# Autodesk Inventor assembly: KS-14_SLow_10inch
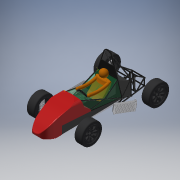
[picture p0: Inventor's stored thumbnail of the model, 180x180]
Saved by Autodesk Inventor 2018.1 (Build 221171000, 171)
## iProperties
Created: 2017-10-13
Part Number: KS-14_SLow_10inch
Material: 一般
Document SubType Name: Assembly
Designer: kuwano
Sending System: Autodesk Inventor 2018
Preprocessor: ST-DEVELOPER v16.13
Title: D:\kuwano\Documents\Inventor\KITformula\CFD_KS-14\KS-14\stl\final_assembly_2017_SuperUltraLow.stp
Author: kuwano
## Documents named in this file (15)
- D:\kuwano\Documents\Inventor\KITformula\KS-15_Aero_CAD\ks-14_slow\KS-14_SLow_10inch.iam
- D:\kuwano\Documents\Inventor\KITformula\KS-15_Aero_CAD\KS-14_SLow\parts\frame3kaiseki_retutch.ipt
- D:\kuwano\Documents\Inventor\KITformula\KS-15_Aero_CAD\KS-14_SLow\parts\F-Upright.iam
- D:\kuwano\Documents\Inventor\KITformula\KS-15_Aero_CAD\KS-14_SLow\parts\R-Upright.iam
- D:\kuwano\Documents\Inventor\KITformula\KS-15_Aero_CAD\KS-14_SLow\parts\driver.ipt
- D:\kuwano\Documents\Inventor\KITformula\KS-15_Aero_CAD\KS-14_SLow\parts\steering assembly.iam
- D:\kuwano\Documents\Inventor\KITformula\KS-15_Aero_CAD\KS-14_SLow\parts\F-Upright_MIR1.iam
- D:\kuwano\Documents\Inventor\KITformula\KS-15_Aero_CAD\KS-14_SLow\parts\R-Upright_MIR2.iam
- D:\kuwano\Documents\Inventor\KITformula\KS-15_Aero_CAD\KS-14_SLow\parts\2017 exhaust assembly_retouch.ipt
- D:\kuwano\Documents\Inventor\KITformula\KS-15_Aero_CAD\KS-14_SLow\parts\kaul_reretouch.ipt
- D:\kuwano\Documents\Inventor\KITformula\KS-15_Aero_CAD\KS-14_SLow\parts\newbody.ipt
- D:\kuwano\Documents\Inventor\KITformula\KS-15_Aero_CAD\KS-14_SLow\parts\radiator 2014 kaiseki.ipt
- D:\kuwano\Documents\Inventor\KITformula\KS-15_Aero_CAD\KS-14_SLow\parts\wall.ipt
- D:\kuwano\Documents\Inventor\KITformula\KS-15_Aero_CAD\KS-14_SLow\parts\wall_MIR1.ipt
- D:\kuwano\Documents\Inventor\KITformula\KS-14\parts\2015Wheel watanabe.ipt
## Components (17 placed, 14 different names)
1. frame3kaiseki_retutch:1 — メイト:2, メイト:3, メイト:4, メイト:5, メイト:6
2. F-Upright:1 [sub-assembly]
3. R-Upright:1 [sub-assembly]
4. driver:1
5. steering assembly:1 [sub-assembly]
6. F-Upright_MIR1:1 [sub-assembly]
7. R-Upright_MIR2:1 [sub-assembly]
8. 2017 exhaust assembly_retouch:1
9. kaul_reretouch:1 — メイト:1
10. newbody:1 — メイト:1
11. radiator 2014 kaiseki:1
12. wall:1 — フラッシュ:1, フラッシュ:2, フラッシュ:3, メイト:2, メイト:3, メイト:4, メイト:5, メイト:6
13. wall_MIR1:1 — メイト:7, メイト:8, フラッシュ:4
14. 2015Wheel watanabe:1
15. 2015Wheel watanabe:2
16. 2015Wheel watanabe:3
17. 2015Wheel watanabe:4
## Relationships (12: Mate 8, Flush 4)
- メイト:1 [Mate]: kaul_reretouch:1 ↔ newbody:1
- フラッシュ:1 [Flush]: wall:1
- フラッシュ:2 [Flush]: wall:1
- フラッシュ:3 [Flush]: wall:1
- メイト:2 [Mate]: frame3kaiseki_retutch:1 ↔ wall:1
- メイト:3 [Mate]: frame3kaiseki_retutch:1 ↔ wall:1
- メイト:4 [Mate]: frame3kaiseki_retutch:1 ↔ wall:1
- メイト:5 [Mate]: frame3kaiseki_retutch:1 ↔ wall:1
- メイト:6 [Mate]: frame3kaiseki_retutch:1 ↔ wall:1
- メイト:7 [Mate]: wall_MIR1:1
- メイト:8 [Mate]: wall_MIR1:1
- フラッシュ:4 [Flush]: wall_MIR1:1
